# Autodesk Inventor assembly: Подставка
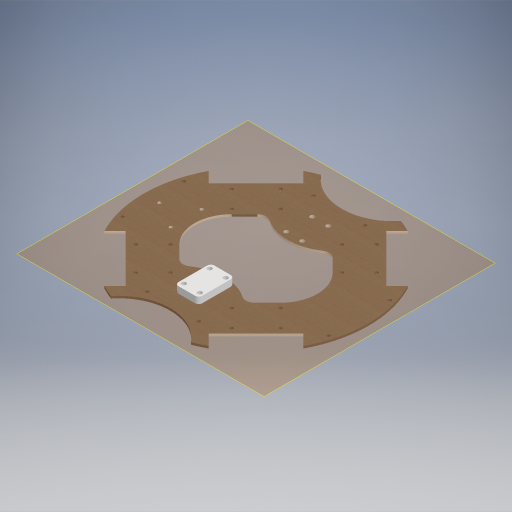
[picture p0: Inventor's stored thumbnail of the model, 512x512]
Saved by Autodesk Inventor 2023 (Build 270158000, 158)
## iProperties
Created: 2025-04-10
Part Number: Подставка
Document SubType Name: Assembly
Designer: Ivan
Author: Ivan
## Documents named in this file (3)
- C:\!projects\DASH-\3D\Dash-V1\Solenoid\Подставка.iam
- C:\!projects\DASH-\3D\Dash-V1\floor_v3.ipt
- C:\!projects\DASH-\3D\Dash-V1\Solenoid\Подставка под солноид.ipt
## Components (2 placed, 2 different names)
1. floor_v3:1 — Заподлицо:1, Заподлицо:2
2. Подставка под солноид:1 — Заподлицо:1, Заподлицо:2
## Relationships (2: Flush 2)
- Заподлицо:1 [Flush]: floor_v3:1 ↔ Подставка под солноид:1
- Заподлицо:2 [Flush]: floor_v3:1 ↔ Подставка под солноид:1
